# Autodesk Inventor assembly: Wheel Module
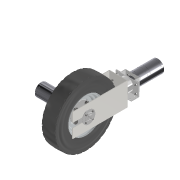
[picture p0: Inventor's stored thumbnail of the model, 180x180]
Saved by Autodesk Inventor 2022 (Build 260153000, 153)
## iProperties
Created: 2024-07-01
Part Number: Wheel Module
Document SubType Name: Assembly
Designer: LaptopJR
Author: LaptopJR
## Documents named in this file (24)
- C:\Users\LaptopJR\Documents\Ideation AI\EcoTerrabot\Chassis\CAD files\Wheel module\Wheel Module.iam
- C:\Users\LaptopJR\Documents\Ideation AI\EcoTerrabot\Chassis\CAD files\Wheel module\PA_402_4_G15.ipt
- C:\Users\LaptopJR\Documents\Ideation AI\EcoTerrabot\Chassis\CAD files\Wheel module\wheelFlange.ipt
- C:\Users\LaptopJR\Documents\Ideation AI\EcoTerrabot\Chassis\CAD files\Wheel module\wheelFlangeMotor.ipt
- C:\Users\LaptopJR\Documents\Ideation AI\EcoTerrabot\Chassis\CAD files\Wheel module\PL82Z-BL82.106-i3.65.ipt
- C:\Users\LaptopJR\Documents\Ideation AI\EcoTerrabot\Chassis\CAD files\Wheel module\Guide Pin.ipt
- C:\Users\LaptopJR\Documents\Ideation AI\EcoTerrabot\Chassis\CAD files\Wheel module\CShape.ipt
- C:\Users\LaptopJR\Documents\Ideation AI\EcoTerrabot\Chassis\CAD files\Wheel module\BearingHolder.ipt
- C:\Users\LaptopJR\Documents\Ideation AI\EcoTerrabot\Chassis\CAD files\Wheel module\Bearing 61806\skf_bearing_61806-2rs1_2.iam
- C:\Users\LaptopJR\Documents\Ideation AI\EcoTerrabot\Chassis\CAD files\Wheel module\MotorBracket.ipt
- C:\Users\LaptopJR\Documents\Inventor\Content Center Files\R2022\en-US\DIN 934\DIN 934 - M6 x 1.ipt
- C:\Users\LaptopJR\Documents\Inventor\Content Center Files\R2022\en-US\SS-ISO 4762\ISO 4762 - M6 x 16SS-ISO.ipt
- C:\Users\LaptopJR\Documents\Inventor\Content Center Files\R2022\en-US\DIN 934\DIN 934 - M5 x 0.8.ipt
- C:\Users\LaptopJR\Documents\Inventor\Content Center Files\R2022\en-US\SS-ISO 4762\ISO 4762 - M5 x 16SS-ISO.ipt
- C:\Users\LaptopJR\Documents\Inventor\Content Center Files\R2022\en-US\ANSI B18.2.1(3)\ANSI B18.2.1 - 9_16-12 UNC - 1.5(3).ipt
- C:\Users\LaptopJR\Documents\Inventor\Content Center Files\R2022\en-US\ANSI B18.2.2(09)\ANSI B18.2.2 - 9_16 - 12(2).ipt
- C:\Users\LaptopJR\Documents\Ideation AI\EcoTerrabot\Chassis\CAD files\Wheel module\wheelFlangeTopMotor.ipt
- C:\Users\LaptopJR\Documents\Ideation AI\EcoTerrabot\Chassis\CAD files\Wheel module\WheelHolder.ipt
- C:\Users\LaptopJR\Documents\Ideation AI\EcoTerrabot\Chassis\CAD files\Wheel module\WheelHolder_S1.ipt
- C:\Users\LaptopJR\Documents\Ideation AI\EcoTerrabot\Chassis\CAD files\Wheel module\WheelHolder_S2.ipt
- C:\Users\LaptopJR\Documents\Ideation AI\EcoTerrabot\Chassis\CAD files\Wheel module\bearing 6306 2rs1\skf_bearing_6306-2rs1_2.iam
- C:\Users\LaptopJR\Documents\Inventor\Content Center Files\R2022\en-US\ANSI AFBMA  8.1 KM\ANSI_AFBMA Std 8.1 - KM 6.ipt
- C:\Users\LaptopJR\Documents\Ideation AI\EcoTerrabot\Chassis\CAD files\Wheel module\bearing 51106\skf_bearing_51106_2.iam
- C:\Users\LaptopJR\Documents\Ideation AI\EcoTerrabot\Chassis\CAD files\Wheel module\TopMotorBracket.ipt
## Components (78 placed, 23 different names)
1. PA_402_4_G15:1 — Mate:1, Mate:2, Mate:3, Mate:4, Mate:5, Mate:6
2. wheelFlange:1 — Mate:1, Mate:2, Mate:6, Mate:10, Mate:23, Insert:8
3. wheelFlangeMotor:1 — Mate:3, Mate:4, Mate:5, Mate:7, Mate:8, Mate:9, Flush:1, Mate:21, Mate:25, Mate:45
4. PL82Z-BL82.106-i3.65:1 — Mate:7, Mate:8, Mate:33, Mate:34, Mate:35
5. Guide Pin:1 — Mate:9, Flush:1
6. CShape:1 — Mate:10, Mate:21, Mate:24, Mate:26, Mate:28, Mate:31, Mate:36, Mate:37, Mate:39, Mate:41, Mate:43, Mate:46, Mate:50, Mate:51, Insert:10
7. BearingHolder:1 — Mate:27, Mate:28, Mate:29, Insert:7
8. BearingHolder:2 — Mate:30, Mate:31, Mate:32, Insert:6
9. skf_bearing_61806-2rs1_2:1 [sub-assembly] — Mate:25, Mate:26, Mate:30, Mate:32
10. skf_bearing_61806-2rs1_2:2 [sub-assembly] — Mate:23, Mate:24, Mate:27, Mate:29
11. MotorBracket:1 — Mate:33, Mate:34, Mate:35, Mate:36, Mate:37, Insert:1, Insert:2, Insert:3, Insert:4, Insert:5
12. SS ISO 4762 M6 x 16:5 — Insert:1
13. SS ISO 4762 M6 x 16:6 — Insert:2
14. SS ISO 4762 M6 x 16:7 — Insert:3
15. SS ISO 4762 M6 x 16:8 — Insert:4
16. wheelFlangeTopMotor:1 — Mate:46, Mate:48, Mate:49, Mate:50, Mate:51, Insert:9, Mate:55, Mate:56, Mate:59, Mate:62, Mate:63, Mate:64, Mate:71, Mate:72, Mate:75
17. PL82Z-BL82.106-i3.65:2 — Mate:48, Mate:49, Mate:54, Mate:76, Mate:77
18. WheelHolder:1 — Mate:54, Mate:69, Mate:73, Mate:78, Mate:79, Mate:81
19. WheelHolder_S1:1 — Mate:55, Mate:56, Mate:65
20. WheelHolder_S2:1 — Mate:59, Mate:67, Mate:68
21. WheelHolder_S1:2 — Mate:62, Mate:66, Mate:69
22. skf_bearing_6306-2rs1_2:1 [sub-assembly] — Mate:63, Mate:65, Mate:68
23. skf_bearing_6306-2rs1_2:2 [sub-assembly] — Mate:64, Mate:66, Mate:67
24. ANSI/AFBMA Std 8.1 KM (Metric) KM 6:1 — Mate:71, Mate:74
25. skf_bearing_51106_2:1 [sub-assembly] — Mate:72, Mate:73, Mate:74
26. TopMotorBracket:1 — Mate:75, Mate:76, Mate:77, Insert:11, Insert:12, Insert:13, Insert:14, Mate:78, Mate:79, Insert:18
27. SS ISO 4762 M6 x 16:13 — Insert:11
28. SS ISO 4762 M6 x 16:14 — Insert:12
29. SS ISO 4762 M6 x 16:15 — Insert:13
30. SS ISO 4762 M6 x 16:16 — Insert:14
31. SS ISO 4762 M6 x 16:1 — Insert:5, Mate:38
32. DIN 934 - replaced by DIN EN 24032/28673/28674 M6:1 — Mate:38, Mate:39
33. SS ISO 4762 M6 x 16:2
34. DIN 934 - replaced by DIN EN 24032/28673/28674 M6:2
35. SS ISO 4762 M6 x 16:3
36. DIN 934 - replaced by DIN EN 24032/28673/28674 M6:3
37. SS ISO 4762 M6 x 16:4
38. DIN 934 - replaced by DIN EN 24032/28673/28674 M6:4
39. SS ISO 4762 M5 x 16:1 — Insert:6, Mate:40
40. DIN 934 - replaced by DIN EN 24032/28673/28674 M5:1 — Mate:40, Mate:41
41. SS ISO 4762 M5 x 16:2
42. DIN 934 - replaced by DIN EN 24032/28673/28674 M5:2
43. SS ISO 4762 M5 x 16:3
44. DIN 934 - replaced by DIN EN 24032/28673/28674 M5:3
45. SS ISO 4762 M5 x 16:4
46. DIN 934 - replaced by DIN EN 24032/28673/28674 M5:4
47. SS ISO 4762 M5 x 16:5 — Insert:7, Mate:42
48. DIN 934 - replaced by DIN EN 24032/28673/28674 M5:5 — Mate:42, Mate:43
49. SS ISO 4762 M5 x 16:6
50. DIN 934 - replaced by DIN EN 24032/28673/28674 M5:6
51. SS ISO 4762 M5 x 16:7
52. DIN 934 - replaced by DIN EN 24032/28673/28674 M5:7
53. SS ISO 4762 M5 x 16:8
54. DIN 934 - replaced by DIN EN 24032/28673/28674 M5:8
55. Hex Cap Screw - Inch 9/16-12 UNC - 1.5:1 — Insert:8, Mate:44
56. Hex Nut - Inch 9/16 - 12:1 — Mate:44, Mate:45
57. Hex Cap Screw - Inch 9/16-12 UNC - 1.5:2
58. Hex Nut - Inch 9/16 - 12:2
59. Hex Cap Screw - Inch 9/16-12 UNC - 1.5:3
60. Hex Nut - Inch 9/16 - 12:3
61. Hex Cap Screw - Inch 9/16-12 UNC - 1.5:4
62. Hex Nut - Inch 9/16 - 12:4
63. SS ISO 4762 M6 x 16:9 — Insert:9
64. DIN 934 - replaced by DIN EN 24032/28673/28674 M6:5 — Insert:10
65. SS ISO 4762 M6 x 16:10
66. DIN 934 - replaced by DIN EN 24032/28673/28674 M6:6
67. SS ISO 4762 M6 x 16:11
68. DIN 934 - replaced by DIN EN 24032/28673/28674 M6:7
69. SS ISO 4762 M6 x 16:12
70. DIN 934 - replaced by DIN EN 24032/28673/28674 M6:8
71. SS ISO 4762 M6 x 16:20 — Insert:18, Mate:80
72. DIN 934 - replaced by DIN EN 24032/28673/28674 M6:9 — Mate:80, Mate:81
73. SS ISO 4762 M6 x 16:21
74. DIN 934 - replaced by DIN EN 24032/28673/28674 M6:10
75. SS ISO 4762 M6 x 16:22
76. DIN 934 - replaced by DIN EN 24032/28673/28674 M6:11
77. SS ISO 4762 M6 x 16:23
78. DIN 934 - replaced by DIN EN 24032/28673/28674 M6:12
## Component patterns: (4 elements, first: SS ISO 4762 M6 x 16:1 + DIN 934 - replaced by DIN EN 24032/28673/28674 M6:1), (4 elements, first: SS ISO 4762 M5 x 16:1 + DIN 934 - replaced by DIN EN 24032/28673/28674 M5:1), (4 elements, first: SS ISO 4762 M5 x 16:5 + DIN 934 - replaced by DIN EN 24032/28673/28674 M5:5), (4 elements, first: Hex Cap Screw - Inch 9/16-12 UNC - 1.5:1 + Hex Nut - Inch 9/16 - 12:1), (4 elements, first: SS ISO 4762 M6 x 16:9 + DIN 934 - replaced by DIN EN 24032/28673/28674 M6:5), (4 elements, first: SS ISO 4762 M6 x 16:20 + DIN 934 - replaced by DIN EN 24032/28673/28674 M6:9)
## Relationships (79: Mate 62, Insert 15, Flush 2)
- Mate:1: PA_402_4_G15:1 ↔ wheelFlange:1
- Mate:2: PA_402_4_G15:1 ↔ wheelFlange:1
- Mate:3 (4 mm): PA_402_4_G15:1 ↔ wheelFlangeMotor:1
- Mate:4: PA_402_4_G15:1 ↔ wheelFlangeMotor:1
- Mate:5: PA_402_4_G15:1 ↔ wheelFlangeMotor:1
- Mate:6 (1 mm): PA_402_4_G15:1 ↔ wheelFlange:1
- Mate:7: wheelFlangeMotor:1 ↔ PL82Z-BL82.106-i3.65:1
- Mate:8: wheelFlangeMotor:1 ↔ PL82Z-BL82.106-i3.65:1
- Mate:9: wheelFlangeMotor:1 ↔ Guide Pin:1
- Flush:1 (40 mm): wheelFlangeMotor:1 ↔ Guide Pin:1
- Mate:10: wheelFlange:1 ↔ CShape:1
- Flush:2 (-200 mm)
- Mate:21 (45 mm): wheelFlangeMotor:1 ↔ CShape:1
- Mate:23: wheelFlange:1 ↔ skf_bearing_61806-2rs1_2:2
- Mate:24: CShape:1 ↔ skf_bearing_61806-2rs1_2:2
- Mate:25: wheelFlangeMotor:1 ↔ skf_bearing_61806-2rs1_2:1
- Mate:26: CShape:1 ↔ skf_bearing_61806-2rs1_2:1
- Mate:27: BearingHolder:1 ↔ skf_bearing_61806-2rs1_2:2
- Mate:28: CShape:1 ↔ BearingHolder:1
- Mate:29: BearingHolder:1 ↔ skf_bearing_61806-2rs1_2:2
- Mate:30: BearingHolder:2 ↔ skf_bearing_61806-2rs1_2:1
- Mate:31: CShape:1 ↔ BearingHolder:2
- Mate:32: BearingHolder:2 ↔ skf_bearing_61806-2rs1_2:1
- Mate:33: PL82Z-BL82.106-i3.65:1 ↔ MotorBracket:1
- Mate:34: PL82Z-BL82.106-i3.65:1 ↔ MotorBracket:1
- Mate:35: PL82Z-BL82.106-i3.65:1 ↔ MotorBracket:1
- Mate:36: CShape:1 ↔ MotorBracket:1
- Mate:37: CShape:1 ↔ MotorBracket:1
- Insert:1: MotorBracket:1 ↔ SS ISO 4762 M6 x 16:5
- Insert:2: MotorBracket:1 ↔ SS ISO 4762 M6 x 16:6
- Insert:3: MotorBracket:1 ↔ SS ISO 4762 M6 x 16:7
- Insert:4: MotorBracket:1 ↔ SS ISO 4762 M6 x 16:8
- Insert:5: MotorBracket:1 ↔ SS ISO 4762 M6 x 16:1
- Mate:38: SS ISO 4762 M6 x 16:1 ↔ DIN 934 - replaced by DIN EN 24032/28673/28674 M6:1
- Mate:39: CShape:1 ↔ DIN 934 - replaced by DIN EN 24032/28673/28674 M6:1
- Insert:6: BearingHolder:2 ↔ SS ISO 4762 M5 x 16:1
- Mate:40: SS ISO 4762 M5 x 16:1 ↔ DIN 934 - replaced by DIN EN 24032/28673/28674 M5:1
- Mate:41: CShape:1 ↔ DIN 934 - replaced by DIN EN 24032/28673/28674 M5:1
- Insert:7: BearingHolder:1 ↔ SS ISO 4762 M5 x 16:5
- Mate:42: SS ISO 4762 M5 x 16:5 ↔ DIN 934 - replaced by DIN EN 24032/28673/28674 M5:5
- Mate:43: CShape:1 ↔ DIN 934 - replaced by DIN EN 24032/28673/28674 M5:5
- Insert:8: wheelFlange:1 ↔ Hex Cap Screw - Inch 9/16-12 UNC - 1.5:1
- Mate:44: Hex Cap Screw - Inch 9/16-12 UNC - 1.5:1 ↔ Hex Nut - Inch 9/16 - 12:1
- Mate:45: wheelFlangeMotor:1 ↔ Hex Nut - Inch 9/16 - 12:1
- Mate:46: CShape:1 ↔ wheelFlangeTopMotor:1
- Mate:48: wheelFlangeTopMotor:1 ↔ PL82Z-BL82.106-i3.65:2
- Mate:49: wheelFlangeTopMotor:1 ↔ PL82Z-BL82.106-i3.65:2
- Mate:50: CShape:1 ↔ wheelFlangeTopMotor:1
- Mate:51: CShape:1 ↔ wheelFlangeTopMotor:1
- Insert:9: wheelFlangeTopMotor:1 ↔ SS ISO 4762 M6 x 16:9
- Insert:10: CShape:1 ↔ DIN 934 - replaced by DIN EN 24032/28673/28674 M6:5
- Mate:54: PL82Z-BL82.106-i3.65:2 ↔ WheelHolder:1
- Mate:55: wheelFlangeTopMotor:1 ↔ WheelHolder_S1:1
- Mate:56: wheelFlangeTopMotor:1 ↔ WheelHolder_S1:1
- Mate:59: wheelFlangeTopMotor:1 ↔ WheelHolder_S2:1
- Mate:62: wheelFlangeTopMotor:1 ↔ WheelHolder_S1:2
- Mate:63: wheelFlangeTopMotor:1 ↔ skf_bearing_6306-2rs1_2:1
- Mate:64: wheelFlangeTopMotor:1 ↔ skf_bearing_6306-2rs1_2:2
- Mate:65: WheelHolder_S1:1 ↔ skf_bearing_6306-2rs1_2:1
- Mate:66: WheelHolder_S1:2 ↔ skf_bearing_6306-2rs1_2:2
- Mate:67: WheelHolder_S2:1 ↔ skf_bearing_6306-2rs1_2:2
- Mate:68: WheelHolder_S2:1 ↔ skf_bearing_6306-2rs1_2:1
- Mate:69: WheelHolder:1 ↔ WheelHolder_S1:2
- Mate:71: wheelFlangeTopMotor:1 ↔ ANSI/AFBMA Std 8.1 KM (Metric) KM 6:1
- Mate:72: wheelFlangeTopMotor:1 ↔ skf_bearing_51106_2:1
- Mate:73: WheelHolder:1 ↔ skf_bearing_51106_2:1
- Mate:74: ANSI/AFBMA Std 8.1 KM (Metric) KM 6:1 ↔ skf_bearing_51106_2:1
- Mate:75: wheelFlangeTopMotor:1 ↔ TopMotorBracket:1
- Mate:76: PL82Z-BL82.106-i3.65:2 ↔ TopMotorBracket:1
- Mate:77: PL82Z-BL82.106-i3.65:2 ↔ TopMotorBracket:1
- Insert:11: TopMotorBracket:1 ↔ SS ISO 4762 M6 x 16:13
- Insert:12: TopMotorBracket:1 ↔ SS ISO 4762 M6 x 16:14
- Insert:13: TopMotorBracket:1 ↔ SS ISO 4762 M6 x 16:15
- Insert:14: TopMotorBracket:1 ↔ SS ISO 4762 M6 x 16:16
- Mate:78: WheelHolder:1 ↔ TopMotorBracket:1
- Mate:79: WheelHolder:1 ↔ TopMotorBracket:1
- Insert:18: TopMotorBracket:1 ↔ SS ISO 4762 M6 x 16:20
- Mate:80: SS ISO 4762 M6 x 16:20 ↔ DIN 934 - replaced by DIN EN 24032/28673/28674 M6:9
- Mate:81: WheelHolder:1 ↔ DIN 934 - replaced by DIN EN 24032/28673/28674 M6:9
